# Autodesk Inventor assembly: X-axis Idler 2 assy
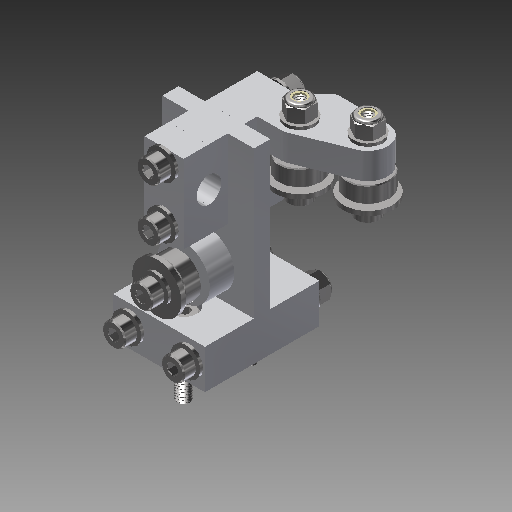
[picture p0: Inventor's stored thumbnail of the model, 512x512]
Saved by Autodesk Inventor 2018 (Build 220112000, 112)
## iProperties
Created: 2017-10-03
Part Number: X-axis Idler 2 assy
Document SubType Name: Assembly
Designer: Gabriel Smolnycki
Author: Gabriel Smolnycki
## Documents named in this file (12)
- E:\planb\mechanics\Subassemblies\X-axis Idler 2 assy.iam
- E:\planb\mechanics\X-axis\X-axis Idler.ipt
- E:\planb\mechanics\X-axis\X-axis Rod Holder.ipt
- E:\planb\mechanics\Hardware\M4 SS Washer.ipt
- E:\planb\mechanics\Hardware\M4 SS Locknut.ipt
- E:\planb\mechanics\Hardware\M4x30 SS SHCS.ipt
- E:\planb\mechanics\X-axis\X-axis Holder Coupler.ipt
- E:\planb\mechanics\Hardware\M4x20 SS SHCS.ipt
- E:\planb\mechanics\Hardware\M4x40 SS SHCS.ipt
- E:\planb\mechanics\Hardware\M5 SS Fender Washer.ipt
- E:\planb\mechanics\Hardware\4x13 SS Ball Bearing (7804K103).ipt
- E:\planb\mechanics\X-axis\X-axis Y Idler.ipt
## Components (47 placed, 11 different names)
1. X-axis Idler:1 — Insert:1, Insert:2, Insert:11, Insert:12, Insert:13, Insert:14, Insert:25, Insert:26, Insert:33, Insert:34
2. X-axis Rod Holder:1 — Insert:1, Insert:2, Insert:3, Insert:4
3. M4 SS Washer:1 — Insert:3
4. M4 SS Washer:2 — Insert:4
5. M4 SS Washer:3 — Insert:7, Insert:35
6. M4 SS Washer:4 — Insert:8, Insert:36
7. M4 SS Locknut:1 — Insert:7
8. M4 SS Locknut:2 — Insert:8
9. M4x40 SS SHCS:3
10. M4x40 SS SHCS:4
11. X-axis Holder Coupler:1 — Insert:11, Insert:12, Insert:16, Insert:19, Insert:20
12. X-axis Holder Coupler:2 — Insert:13, Insert:14, Insert:15, Insert:17, Insert:18
13. M4x20 SS SHCS:1 — Insert:16
14. M4x20 SS SHCS:2 — Insert:15
15. M4 SS Washer:5 — Insert:17, Insert:23
16. M4 SS Washer:6 — Insert:18, Insert:24
17. M4 SS Washer:7 — Insert:19, Insert:22
18. M4 SS Washer:8 — Insert:20, Insert:21
19. M4 SS Locknut:3 — Insert:21
20. M4 SS Locknut:4 — Insert:22
21. M4x40 SS SHCS:1 — Insert:23
22. M4x40 SS SHCS:2 — Insert:24
23. M4 SS Washer:9 — Insert:25, Insert:31
24. M4 SS Washer:10 — Insert:26, Insert:27
25. M4 SS Washer:11 — Insert:28, Insert:29
26. M4 SS Washer:12 — Insert:30, Insert:32
27. M5 SS Fender Washer:1 — Insert:29, Insert:30
28. 4x13 SS Ball Bearing (7804K103):1 — Insert:27, Insert:28
29. M4 SS Locknut:5 — Insert:31
30. M4x30 SS SHCS:3 — Insert:32
31. X-axis Y Idler:1 — Insert:33, Insert:34, Insert:35, Insert:36, Insert:37, Insert:38, Insert:51, Insert:52
32. M4 SS Washer:13 — Insert:38, Insert:40
33. M4 SS Washer:14 — Insert:37, Insert:39
34. M4 SS Locknut:6 — Insert:40
35. M4 SS Locknut:7 — Insert:39
36. M4x20 SS SHCS:3 — Insert:41
37. M4 SS Washer:15 — Insert:41, Insert:42
38. M4 SS Washer:16 — Insert:43, Insert:44
39. M4 SS Washer:17 — Insert:45, Insert:51
40. M5 SS Fender Washer:2 — Insert:42, Insert:43
41. 4x13 SS Ball Bearing (7804K103):2 — Insert:44, Insert:45
42. M4x20 SS SHCS:4
43. M4 SS Washer:18
44. M4 SS Washer:19
45. M4 SS Washer:20 — Insert:52
46. M5 SS Fender Washer:3
47. 4x13 SS Ball Bearing (7804K103):3
## Relationships (50: Insert 50)
- Insert:1: X-axis Idler:1 ↔ X-axis Rod Holder:1
- Insert:2: X-axis Idler:1 ↔ X-axis Rod Holder:1
- Insert:3: X-axis Rod Holder:1 ↔ M4 SS Washer:1
- Insert:4: X-axis Rod Holder:1 ↔ M4 SS Washer:2
- Insert:7: M4 SS Washer:3 ↔ M4 SS Locknut:1
- Insert:8: M4 SS Washer:4 ↔ M4 SS Locknut:2
- [Insert]: M4 SS Washer:1 ↔ M4x40 SS SHCS:3
- [Insert]: M4 SS Washer:2 ↔ M4x40 SS SHCS:4
- Insert:11: X-axis Idler:1 ↔ X-axis Holder Coupler:1
- Insert:12: X-axis Idler:1 ↔ X-axis Holder Coupler:1
- Insert:13: X-axis Idler:1 ↔ X-axis Holder Coupler:2
- Insert:14: X-axis Idler:1 ↔ X-axis Holder Coupler:2
- Insert:15: X-axis Holder Coupler:2 ↔ M4x20 SS SHCS:2
- Insert:16: X-axis Holder Coupler:1 ↔ M4x20 SS SHCS:1
- Insert:17: X-axis Holder Coupler:2 ↔ M4 SS Washer:5
- Insert:18: X-axis Holder Coupler:2 ↔ M4 SS Washer:6
- Insert:19: X-axis Holder Coupler:1 ↔ M4 SS Washer:7
- Insert:20: X-axis Holder Coupler:1 ↔ M4 SS Washer:8
- Insert:21: M4 SS Washer:8 ↔ M4 SS Locknut:3
- Insert:22: M4 SS Washer:7 ↔ M4 SS Locknut:4
- Insert:23: M4 SS Washer:5 ↔ M4x40 SS SHCS:1
- Insert:24: M4 SS Washer:6 ↔ M4x40 SS SHCS:2
- Insert:25: X-axis Idler:1 ↔ M4 SS Washer:9
- Insert:26: X-axis Idler:1 ↔ M4 SS Washer:10
- Insert:27: M4 SS Washer:10 ↔ 4x13 SS Ball Bearing (7804K103):1
- Insert:28: M4 SS Washer:11 ↔ 4x13 SS Ball Bearing (7804K103):1
- Insert:29: M4 SS Washer:11 ↔ M5 SS Fender Washer:1
- Insert:30: M4 SS Washer:12 ↔ M5 SS Fender Washer:1
- Insert:31: M4 SS Washer:9 ↔ M4 SS Locknut:5
- Insert:32: M4 SS Washer:12 ↔ M4x30 SS SHCS:3
- Insert:33: X-axis Idler:1 ↔ X-axis Y Idler:1
- Insert:34: X-axis Idler:1 ↔ X-axis Y Idler:1
- Insert:35: M4 SS Washer:3 ↔ X-axis Y Idler:1
- Insert:36: M4 SS Washer:4 ↔ X-axis Y Idler:1
- Insert:37: X-axis Y Idler:1 ↔ M4 SS Washer:14
- Insert:38: X-axis Y Idler:1 ↔ M4 SS Washer:13
- Insert:39: M4 SS Washer:14 ↔ M4 SS Locknut:7
- Insert:40: M4 SS Washer:13 ↔ M4 SS Locknut:6
- Insert:41: M4x20 SS SHCS:3 ↔ M4 SS Washer:15
- Insert:42: M4 SS Washer:15 ↔ M5 SS Fender Washer:2
- Insert:43: M4 SS Washer:16 ↔ M5 SS Fender Washer:2
- Insert:44: M4 SS Washer:16 ↔ 4x13 SS Ball Bearing (7804K103):2
- Insert:45: M4 SS Washer:17 ↔ 4x13 SS Ball Bearing (7804K103):2
- [Insert]: M4x20 SS SHCS:4 ↔ M4 SS Washer:18
- [Insert]: M4 SS Washer:18 ↔ M5 SS Fender Washer:3
- [Insert]: M4 SS Washer:19 ↔ M5 SS Fender Washer:3
- [Insert]: M4 SS Washer:19 ↔ 4x13 SS Ball Bearing (7804K103):3
- [Insert]: M4 SS Washer:20 ↔ 4x13 SS Ball Bearing (7804K103):3
- Insert:51: X-axis Y Idler:1 ↔ M4 SS Washer:17
- Insert:52: X-axis Y Idler:1 ↔ M4 SS Washer:20
## Named parameters: d45_d40 = 0 mm, d46_d41 = 0 mm, d47_d42 = 0 mm, d48_d43 = 0 mm, d49_d44 = 0 mm
